# Autodesk Inventor assembly: 25Assembly-0004-OK
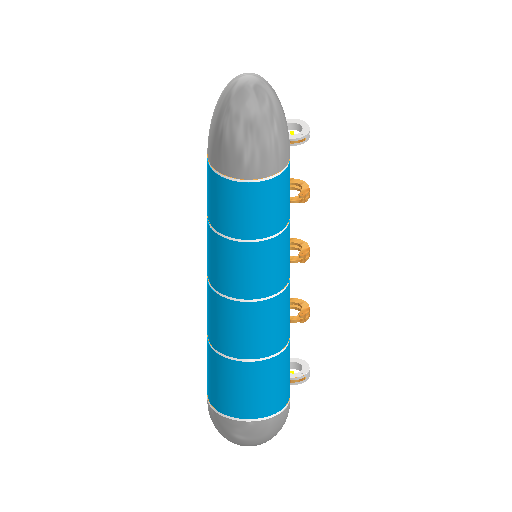
[picture p0: Inventor's stored thumbnail of the model, 512x512]
Saved by Autodesk Inventor 2025.2 (Build 292293000, 293)
## iProperties
Created: 2025-03-09
Part Number: 25Assembly-0004-OK
Document SubType Name: Assembly
Designer: Oscar
Author: Oscar
## Documents named in this file (16)
- C:\Users\alexb\Downloads\Pod CAD - Copy\A01v14.iam
- C:\Users\alexb\Downloads\Pod CAD - Copy\P06.01.ipt
- C:\Users\alexb\Downloads\Pod CAD - Copy\P01.02.ipt
- C:\Users\alexb\Downloads\Pod CAD - Copy\P01.01.ipt
- C:\Users\alexb\Downloads\Pod CAD - Copy\P02.01.ipt
- C:\Users\alexb\Downloads\Pod CAD - Copy\P07.01.ipt
- C:\Users\alexb\Downloads\Pod CAD - Copy\P07.02.ipt
- C:\Users\alexb\Downloads\Pod CAD - Copy\P03.01.ipt
- C:\Users\alexb\Downloads\Pod CAD - Copy\P05.02.ipt
- C:\Users\alexb\Downloads\Pod CAD - Copy\P05.03.ipt
- C:\Users\alexb\Downloads\Pod CAD - Copy\P05.04.ipt
- C:\Users\alexb\Downloads\Pod CAD - Copy\P05.01.ipt
- C:\Users\alexb\Downloads\Pod CAD - Copy\P02.02.ipt
- C:\Users\alexb\Downloads\Pod CAD - Copy\P02.03.ipt
- C:\Users\alexb\Downloads\Pod CAD - Copy\P04.02.ipt
- C:\Users\alexb\Downloads\Pod CAD - Copy\P04.01.ipt
## Components (62 placed, 15 different names)
1. P06.01:1 — Mate:1, Mate:2, Mate:3, Mate:4, Mate:5, Mate:6, Mate:7, Mate:8, Flush:13, Mate:53, Mate:54, Mate:55, Mate:77, Mate:79, Mate:90, Flush:39, Mate:128, Mate:129, Mate:131, Mate:133
2. P01.02:1 — Mate:1, Mate:9, Mate:11, Mate:13, Mate:15, Flush:14, Mate:29, Mate:32, Mate:33, Mate:36
3. P01.02:2 — Mate:2, Mate:10, Mate:12, Mate:14, Mate:16, Flush:15, Mate:30, Mate:31, Mate:34, Mate:35
4. P01.02:3 — Mate:3, Flush:20, Mate:41, Mate:42, Mate:43, Mate:44
5. P01.02:4 — Mate:4, Flush:21, Mate:37, Mate:38, Mate:39, Mate:40
6. P01.01:1 — Mate:5, Flush:18, Mate:49, Mate:50, Mate:51, Mate:52
7. P01.01:2 — Mate:8, Flush:17, Mate:21, Mate:23, Mate:25, Mate:27
8. P01.01:3 — Mate:7, Flush:16, Mate:45, Mate:46, Mate:47, Mate:48, Mate:92, Mate:135
9. P01.01:4 — Mate:6, Flush:19, Mate:22, Mate:24, Mate:26, Mate:28, Mate:93, Mate:136
10. P06.01:2 — Mate:9, Mate:10, Mate:17, Mate:59, Mate:60, Mate:61, Mate:62, Mate:63, Mate:64, Mate:101, Mate:102, Mate:123, Mate:124
11. P06.01:3 — Mate:11, Mate:12, Mate:18, Mate:65, Mate:66, Mate:67, Mate:68, Mate:69, Mate:70, Mate:103, Mate:104, Mate:121, Mate:122
12. P06.01:4 — Mate:13, Mate:14, Mate:19, Mate:71, Mate:72, Mate:73, Mate:74, Mate:75, Mate:76, Mate:105, Mate:106, Mate:119, Mate:120
13. P06.01:5 — Mate:15, Mate:16, Mate:20, Mate:56, Mate:57, Mate:58, Flush:38, Mate:82
14. P02.01:1 — Mate:21, Mate:22, Flush:22, Mate:107, Mate:108, Mate:109
15. P02.01:2 — Mate:23, Mate:24, Flush:23
16. P02.01:3 — Mate:25, Mate:26, Flush:24, Mate:110, Mate:111
17. P02.01:4 — Mate:27, Mate:28, Flush:25, Mate:112
18. P02.01:5 — Mate:35, Mate:36, Flush:29
19. P02.01:6 — Mate:33, Mate:34, Flush:28
20. P02.01:7 — Mate:31, Mate:32, Flush:27
21. P02.01:8 — Mate:29, Mate:30, Flush:26
22. P02.01:9 — Mate:37, Mate:41, Flush:30
23. P02.01:10 — Mate:38, Mate:42, Flush:31
24. P02.01:11 — Mate:39, Mate:43, Flush:32
25. P02.01:12 — Mate:40, Mate:44, Flush:33
26. P02.01:13 — Mate:48, Mate:49, Flush:34, Mate:94
27. P02.01:14 — Mate:47, Mate:50, Flush:35, Mate:95, Mate:96
28. P02.01:15 — Mate:46, Mate:51, Flush:36, Mate:97, Mate:98
29. P02.01:16 — Mate:45, Mate:52, Flush:37, Mate:99, Mate:100
30. P07.01:1 — Mate:53, Mate:54, Mate:55
31. P07.01:2 — Mate:56, Mate:57, Mate:58
32. P07.02:1 — Mate:59, Mate:60, Mate:61
33. P07.02:2 — Mate:62, Mate:63, Mate:64
34. P07.02:3 — Mate:65, Mate:66, Mate:67
35. P07.02:4 — Mate:68, Mate:69, Mate:70
36. P07.02:5 — Mate:71, Mate:72, Mate:73
37. P07.02:6 — Mate:74, Mate:75, Mate:76
38. P03.01:1 — Mate:77, Mate:79, Flush:38, Mate:132, Mate:134
39. P05.02:1 — Mate:82, Mate:86, Mate:87, Mate:88, Mate:89, Mate:92, Mate:93
40. P05.03:1 — Mate:88, Mate:89
41. P05.04:1 — Mate:86, Mate:87
42. P05.01:1 — Mate:90
43. P02.02:1 — Mate:94, Flush:40, Flush:47
44. P02.02:2 — Mate:95, Flush:42, Mate:102
45. P02.02:3 — Mate:97, Flush:44, Mate:104
46. P02.02:4 — Mate:96, Flush:41, Mate:101, Mate:125, Flush:48
47. P02.02:5 — Mate:98, Flush:43, Mate:103
48. P02.02:6 — Mate:99, Flush:46, Mate:106
49. P02.02:7 — Mate:100, Flush:45, Mate:105
50. P02.02:8 — Mate:107, Mate:114, Mate:122
51. P02.02:9 — Mate:108, Mate:115, Mate:120
52. P02.02:10 — Mate:109, Mate:113, Mate:121
53. P02.02:11 — Mate:110, Mate:116, Mate:123
54. P02.02:12 — Mate:111, Mate:117, Mate:124, Mate:126, Flush:49
55. P02.02:13 — Mate:112, Mate:118, Mate:119
56. P02.03:1 — Mate:125, Flush:48
57. P02.03:2 — Mate:126, Flush:49
58. P04.02:1 — Mate:127, Mate:128, Flush:51
59. P04.02:2 — Mate:129, Mate:130, Flush:53, Mate:137
60. P04.02:3 — Mate:131, Mate:132, Flush:55
61. P04.02:4 — Mate:133, Mate:134, Flush:57
62. P04.01:1 — Mate:135, Mate:136, Mate:137
## Relationships (179: Mate 130, Flush 49)
- Mate:1: P06.01:1 ↔ P01.02:1
- Mate:2: P06.01:1 ↔ P01.02:2
- Mate:3: P06.01:1 ↔ P01.02:3
- Mate:4: P06.01:1 ↔ P01.02:4
- Mate:5: P06.01:1 ↔ P01.01:1
- Mate:6: P06.01:1 ↔ P01.01:4
- Mate:7: P06.01:1 ↔ P01.01:3
- Mate:8: P06.01:1 ↔ P01.01:2
- Mate:9: P01.02:1 ↔ P06.01:2
- Mate:10: P01.02:2 ↔ P06.01:2
- Mate:11: P01.02:1 ↔ P06.01:3
- Mate:12: P01.02:2 ↔ P06.01:3
- Mate:13: P01.02:1 ↔ P06.01:4
- Mate:14: P01.02:2 ↔ P06.01:4
- Mate:15: P01.02:1 ↔ P06.01:5
- Mate:16: P01.02:2 ↔ P06.01:5
- Flush:9 (-150 mm)
- Mate:17: P06.01:2
- Flush:10 (-300 mm)
- Flush:11 (-450 mm)
- Flush:12 (-600 mm)
- Flush:13 (3 mm): P06.01:1
- Flush:14: P01.02:1
- Flush:15: P01.02:2
- Flush:16: P01.01:3
- Flush:17: P01.01:2
- Flush:18: P01.01:1
- Flush:19: P01.01:4
- Flush:20: P01.02:3
- Flush:21: P01.02:4
- Mate:18: P06.01:3
- Mate:19: P06.01:4
- Mate:20: P06.01:5
- Mate:21: P01.01:2 ↔ P02.01:1
- Mate:22: P01.01:4 ↔ P02.01:1
- Flush:22: P02.01:1
- Mate:23: P01.01:2 ↔ P02.01:2
- Mate:24: P01.01:4 ↔ P02.01:2
- Flush:23: P02.01:2
- Mate:25: P01.01:2 ↔ P02.01:3
- Mate:26: P01.01:4 ↔ P02.01:3
- Flush:24: P02.01:3
- Mate:27: P01.01:2 ↔ P02.01:4
- Mate:28: P01.01:4 ↔ P02.01:4
- Flush:25: P02.01:4
- Mate:29: P01.02:1 ↔ P02.01:8
- Mate:30: P01.02:2 ↔ P02.01:8
- Flush:26: P02.01:8
- Mate:31: P01.02:2 ↔ P02.01:7
- Mate:32: P01.02:1 ↔ P02.01:7
- Flush:27: P02.01:7
- Mate:33: P01.02:1 ↔ P02.01:6
- Mate:34: P01.02:2 ↔ P02.01:6
- Flush:28: P02.01:6
- Mate:35: P01.02:2 ↔ P02.01:5
- Mate:36: P01.02:1 ↔ P02.01:5
- Flush:29: P02.01:5
- Mate:37: P01.02:4 ↔ P02.01:9
- Mate:38: P01.02:4 ↔ P02.01:10
- Mate:39: P01.02:4 ↔ P02.01:11
- Mate:40: P01.02:4 ↔ P02.01:12
- Mate:41: P01.02:3 ↔ P02.01:9
- Mate:42: P01.02:3 ↔ P02.01:10
- Mate:43: P01.02:3 ↔ P02.01:11
- Mate:44: P01.02:3 ↔ P02.01:12
- Flush:30: P02.01:9
- Flush:31: P02.01:10
- Flush:32: P02.01:11
- Flush:33: P02.01:12
- Mate:45: P01.01:3 ↔ P02.01:16
- Mate:46: P01.01:3 ↔ P02.01:15
- Mate:47: P01.01:3 ↔ P02.01:14
- Mate:48: P01.01:3 ↔ P02.01:13
- Mate:49: P01.01:1 ↔ P02.01:13
- Mate:50: P01.01:1 ↔ P02.01:14
- Mate:51: P01.01:1 ↔ P02.01:15
- Mate:52: P01.01:1 ↔ P02.01:16
- Flush:34: P02.01:13
- Flush:35: P02.01:14
- Flush:36: P02.01:15
- Flush:37: P02.01:16
- Mate:53: P06.01:1 ↔ P07.01:1
- Mate:54: P06.01:1 ↔ P07.01:1
- Mate:55: P06.01:1 ↔ P07.01:1
- Mate:56: P06.01:5 ↔ P07.01:2
- Mate:57: P06.01:5 ↔ P07.01:2
- Mate:58: P06.01:5 ↔ P07.01:2
- Mate:59: P06.01:2 ↔ P07.02:1
- Mate:60: P06.01:2 ↔ P07.02:1
- Mate:61: P06.01:2 ↔ P07.02:1
- Mate:62: P06.01:2 ↔ P07.02:2
- Mate:63: P06.01:2 ↔ P07.02:2
- Mate:64: P06.01:2 ↔ P07.02:2
- Mate:65: P06.01:3 ↔ P07.02:3
- Mate:66: P06.01:3 ↔ P07.02:3
- Mate:67: P06.01:3 ↔ P07.02:3
- Mate:68: P06.01:3 ↔ P07.02:4
- Mate:69: P06.01:3 ↔ P07.02:4
- Mate:70: P06.01:3 ↔ P07.02:4
- Mate:71: P06.01:4 ↔ P07.02:5
- Mate:72: P06.01:4 ↔ P07.02:5
- Mate:73: P06.01:4 ↔ P07.02:5
- Mate:74: P06.01:4 ↔ P07.02:6
- Mate:75: P06.01:4 ↔ P07.02:6
- Mate:76: P06.01:4 ↔ P07.02:6
- Mate:77: P06.01:1 ↔ P03.01:1
- Mate:79: P06.01:1 ↔ P03.01:1
- Flush:38: P06.01:5 ↔ P03.01:1
- Mate:82: P06.01:5 ↔ P05.02:1
- Mate:86: P05.02:1 ↔ P05.04:1
- Mate:87: P05.02:1 ↔ P05.04:1
- Mate:88: P05.02:1 ↔ P05.03:1
- Mate:89: P05.02:1 ↔ P05.03:1
- Mate:90: P06.01:1 ↔ P05.01:1
- Mate:92: P01.01:3 ↔ P05.02:1
- Mate:93: P01.01:4 ↔ P05.02:1
- Flush:39 (42 mm): P06.01:1
- Mate:94: P02.01:13 ↔ P02.02:1
- Mate:95: P02.01:14 ↔ P02.02:2
- Mate:96: P02.01:14 ↔ P02.02:4
- Mate:97: P02.01:15 ↔ P02.02:3
- Mate:98: P02.01:15 ↔ P02.02:5
- Mate:99: P02.01:16 ↔ P02.02:6
- Mate:100: P02.01:16 ↔ P02.02:7
- Flush:40: P02.02:1
- Flush:41: P02.02:4
- Flush:42: P02.02:2
- Flush:43: P02.02:5
- Flush:44: P02.02:3
- Flush:45: P02.02:7
- Flush:46: P02.02:6
- Flush:47: P02.02:1
- Mate:101: P06.01:2 ↔ P02.02:4
- Mate:102: P06.01:2 ↔ P02.02:2
- Mate:103: P06.01:3 ↔ P02.02:5
- Mate:104: P06.01:3 ↔ P02.02:3
- Mate:105: P06.01:4 ↔ P02.02:7
- Mate:106: P06.01:4 ↔ P02.02:6
- Mate:107: P02.01:1 ↔ P02.02:8
- Mate:108: P02.01:1 ↔ P02.02:9
- Mate:109: P02.01:1 ↔ P02.02:10
- Mate:110: P02.01:3 ↔ P02.02:11
- Mate:111: P02.01:3 ↔ P02.02:12
- Mate:112: P02.01:4 ↔ P02.02:13
- Mate:113: P02.02:10
- Mate:114: P02.02:8
- Mate:115: P02.02:9
- Mate:116: P02.02:11
- Mate:117: P02.02:12
- Mate:118: P02.02:13
- Mate:119: P06.01:4 ↔ P02.02:13
- Mate:120: P06.01:4 ↔ P02.02:9
- Mate:121: P06.01:3 ↔ P02.02:10
- Mate:122: P06.01:3 ↔ P02.02:8
- Mate:123: P06.01:2 ↔ P02.02:11
- Mate:124: P06.01:2 ↔ P02.02:12
- Mate:125: P02.02:4 ↔ P02.03:1
- Flush:48 (-5 mm): P02.02:4 ↔ P02.03:1
- Mate:126: P02.02:12 ↔ P02.03:2
- Flush:49 (-5 mm): P02.02:12 ↔ P02.03:2
- Mate:127: P04.02:1
- Mate:128: P06.01:1 ↔ P04.02:1
- Flush:50 (-55 mm)
- Flush:51: P04.02:1
- Flush:52 (-148 mm)
- Mate:129: P06.01:1 ↔ P04.02:2
- Mate:130: P04.02:2
- Flush:53: P04.02:2
- Flush:54 (-75 mm)
- Mate:131: P06.01:1 ↔ P04.02:3
- Mate:132: P03.01:1 ↔ P04.02:3
- Flush:55: P04.02:3
- Flush:56 (75 mm)
- Mate:133: P06.01:1 ↔ P04.02:4
- Mate:134: P03.01:1 ↔ P04.02:4
- Flush:57: P04.02:4
- Mate:135: P01.01:3 ↔ P04.01:1
- Mate:136: P01.01:4 ↔ P04.01:1
- Mate:137: P04.02:2 ↔ P04.01:1
